# Autodesk Inventor assembly: BELT_SUPPORT_INNER
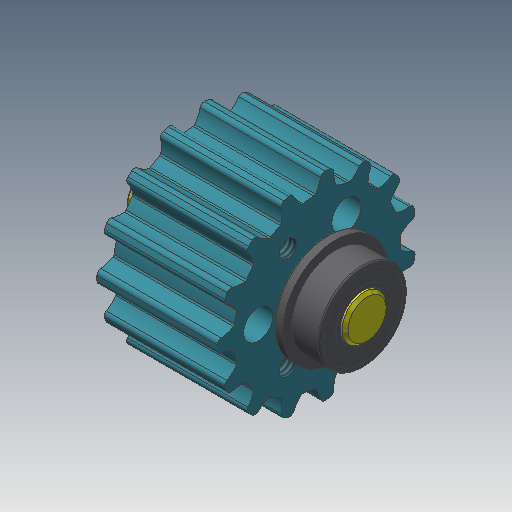
[picture p0: Inventor's stored thumbnail of the model, 512x512]
Saved by Autodesk Inventor 2019.4 (Build 234330000, 330)
## iProperties
Created: 2019-11-12
Part Number: BELT_SUPPORT_INNER
Material: 一般
Document SubType Name: Assembly
Designer: y6tada
Author: y6tada
## Documents named in this file (4)
- C:\Workspace\Yuni9\Inventor\Asm\UPPER_LEG\BELT_SUPPORT_INNER.iam
- C:\Workspace\Yuni9\Inventor\Asm\TIMING_PULLEY\TIMING_BELT_P15.ipt
- C:\Workspace\Yuni9\Inventor\Asm\UPPER_LEG\SHAFT_3x15.ipt
- C:\Workspace\Yuni9\Inventor\Ref\NSK Bearing\NSK_RB_MF63ZZ\MF63ZZ.iam
## Components (3 placed, 3 different names)
1. TIMING_BELT_P15:1 — メイト:1, フラッシュ:1, フラッシュ:2, メイト:2
2. SHAFT_3x15:1 — フラッシュ:3, メイト:2, メイト:3
3. MF63ZZ:1 [sub-assembly] — メイト:3
## Relationships (6: Mate 3, Flush 3)
- メイト:1 [Mate]: TIMING_BELT_P15:1
- フラッシュ:1 [Flush]: TIMING_BELT_P15:1
- フラッシュ:2 [Flush]: TIMING_BELT_P15:1
- フラッシュ:3 [Flush]: SHAFT_3x15:1
- メイト:2 [Mate]: TIMING_BELT_P15:1 ↔ SHAFT_3x15:1
- メイト:3 [Mate]: SHAFT_3x15:1 ↔ MF63ZZ:1
